# Autodesk Inventor assembly: Flex
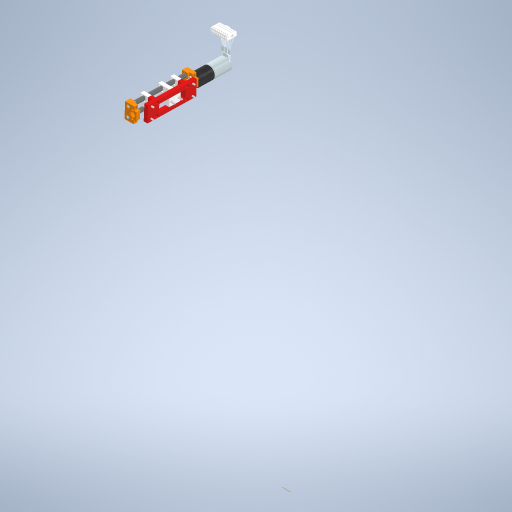
[picture p0: Inventor's stored thumbnail of the model, 512x512]
Saved by Autodesk Inventor 2023 (Build 270158000, 158)
## iProperties
Created: 2023-03-17
Part Number: Flex
Document SubType Name: Assembly
Designer: Nathann
Author: Nathann
## Documents named in this file (23)
- C:\Users\Nathann\ClawdDrive\Objet3D\IminaProbe\V3Roue\DifferentialLinearActuator.iam
- C:\Users\Nathann\OneDrive\ClawdDrive\Objet3D\IminaProbe\V2\Part1.ipt
- C:\Users\Nathann\OneDrive\ClawdDrive\Objet3D\IminaProbe\V2\GP16A_2-Stufig-110322.ipt
- C:\Users\Nathann\OneDrive\ClawdDrive\Objet3D\IminaProbe\V2\283825_ec-max16_5w.ipt
- C:\Users\Nathann\OneDrive\ClawdDrive\Objet3D\IminaProbe\V2\4145N198_Set Screw Precision Flexible Shaft Couplings.ipt
- C:\Users\Nathann\OneDrive\ClawdDrive\Objet3D\IminaProbe\V2\94450A564_Left-Hand Threaded 18-8 Stainless Steel Thin Hex Nut.ipt
- C:\Users\Nathann\OneDrive\ClawdDrive\Objet3D\IminaProbe\V2\91292A832_18-8 Stainless Steel Socket Head Screw.ipt
- C:\Users\Nathann\OneDrive\ClawdDrive\Objet3D\IminaProbe\V2\POMSliderMotor.ipt
- C:\Users\Nathann\OneDrive\ClawdDrive\Objet3D\IminaProbe\V2\MotorMountDifferential.ipt
- C:\Users\Nathann\OneDrive\ClawdDrive\Objet3D\IminaProbe\V2\93805A627_18-8 Stainless Steel Threaded Rod.ipt
- C:\Users\Nathann\OneDrive\ClawdDrive\Objet3D\IminaProbe\V2\93805A631_18-8 Stainless Steel Threaded Rod.ipt
- C:\Users\Nathann\OneDrive\ClawdDrive\Objet3D\IminaProbe\V2\91828A113_18-8 Stainless Steel Hex Nut.ipt
- C:\Users\Nathann\OneDrive\ClawdDrive\Objet3D\IminaProbe\V2\MotorDifferentialMountingBracket.ipt
- C:\Users\Nathann\OneDrive\ClawdDrive\Objet3D\IminaProbe\V2\POMSliderMotorM25.ipt
- C:\Users\Nathann\OneDrive\ClawdDrive\Objet3D\IminaProbe\V2\SliderFixtureM25.ipt
- C:\Users\Nathann\OneDrive\ClawdDrive\Objet3D\IminaProbe\V2\AxisLinear.ipt
- C:\Users\Nathann\OneDrive\ClawdDrive\Objet3D\IminaProbe\V2\POMSliderAxis.ipt
- C:\Users\Nathann\OneDrive\ClawdDrive\Objet3D\IminaProbe\V2\Flex\AIP\FEA\ea0gbbme8.fins
- C:\Users\Nathann\OneDrive\ClawdDrive\Objet3D\IminaProbe\V2\Flex\AIP\FEA\ea0gbbme8.fsat
- C:\Users\Nathann\OneDrive\ClawdDrive\Objet3D\IminaProbe\V2\Flex\AIP\FEA\ea0gbbme8.ftes
- C:\Users\Nathann\OneDrive\ClawdDrive\Objet3D\IminaProbe\V2\Flex\AIP\FEA\ea0gbbme8.fwiz
- C:\Users\Nathann\OneDrive\ClawdDrive\Objet3D\IminaProbe\V2\Flex\AIP\FEA\ea0gbbmf4.fmsh
- C:\Users\Nathann\OneDrive\ClawdDrive\Objet3D\IminaProbe\V2\Flex\AIP\FEA\ea0gbbmf5.fres
## Components (39 placed, 16 different names)
1. Part1:1
2. GP16A_2-Stufig-110322:2 — Insert:23, Insert:24
3. 283825_ec-max16_5w:2
4. 4145N198_Set Screw Precision Flexible Shaft Couplings:2 — Insert:27
5. 91292A832_18-8 Stainless Steel Socket Head Screw:5 — Insert:28
6. 91292A832_18-8 Stainless Steel Socket Head Screw:6 — Insert:29
7. MotorMountDifferential:1 — Insert:23, Insert:24, Insert:28, Insert:29, Flush:10, Flush:12, Flush:13, Insert:43, Insert:44, Insert:45, Insert:46
8. 93805A627_18-8 Stainless Steel Threaded Rod:1 — Insert:26, Rotation:1
9. 93805A631_18-8 Stainless Steel Threaded Rod:2 — Insert:26, Insert:27, Rotation:1
10. 91828A113_18-8 Stainless Steel Hex Nut:1 — Mate:26, Mate:27, Mate:28
11. 94450A564_Left-Hand Threaded 18-8 Stainless Steel Thin Hex Nut:3 — Mate:21, Mate:22, Mate:23
12. MotorDifferentialMountingBracket:1 — Insert:30, Insert:31, Insert:32, Insert:33, Flush:14, Flush:15, Mate:25, Insert:34, Insert:35, Insert:36, Insert:37, Flush:16, Mate:29, Flush:17
13. POMSliderMotorM25:1 — Mate:15, Flush:9, Flush:10, Flush:11, Mate:26, Mate:27, Mate:28, Insert:52, Flush:26
14. SliderFixtureM25:1 — Mate:15, Flush:9, Flush:11, Insert:38, Insert:39, Flush:17
15. POMSliderMotor:3 — Flush:12, Flush:14, Flush:15, Mate:25, Insert:53
16. POMSliderMotor:4 — Flush:13, Mate:21, Mate:22, Mate:23, Flush:16, Mate:29, Insert:51
17. 91292A832_18-8 Stainless Steel Socket Head Screw:9 — Insert:31
18. 91292A832_18-8 Stainless Steel Socket Head Screw:10 — Insert:30
19. 91292A832_18-8 Stainless Steel Socket Head Screw:11 — Insert:33
20. 91292A832_18-8 Stainless Steel Socket Head Screw:12 — Insert:32
21. 91292A832_18-8 Stainless Steel Socket Head Screw:13 — Insert:36
22. 91292A832_18-8 Stainless Steel Socket Head Screw:14 — Insert:34
23. 91292A832_18-8 Stainless Steel Socket Head Screw:15 — Insert:37
24. 91292A832_18-8 Stainless Steel Socket Head Screw:16 — Insert:35
25. 91292A832_18-8 Stainless Steel Socket Head Screw:17 — Insert:39
26. 91292A832_18-8 Stainless Steel Socket Head Screw:18 — Insert:38
27. AxisLinear:1 — Insert:43, Insert:47
28. AxisLinear:2 — Insert:44, Insert:48
29. 91292A832_18-8 Stainless Steel Socket Head Screw:19 — Insert:46
30. 91292A832_18-8 Stainless Steel Socket Head Screw:20 — Insert:45
31. MotorMountDifferential:2 — Insert:47, Insert:48, Insert:49, Insert:50, Flush:18
32. 91292A832_18-8 Stainless Steel Socket Head Screw:21 — Insert:49
33. 91292A832_18-8 Stainless Steel Socket Head Screw:22 — Insert:50
34. POMSliderAxis:1 — Insert:52, Insert:55, Flush:26
35. POMSliderAxis:2 — Insert:53, Insert:56, Flush:18
36. POMSliderAxis:3 — Insert:51, Insert:54
37. 91292A832_18-8 Stainless Steel Socket Head Screw:23 — Insert:56
38. 91292A832_18-8 Stainless Steel Socket Head Screw:24 — Insert:55
39. 91292A832_18-8 Stainless Steel Socket Head Screw:25 — Insert:54
## Relationships (53: Insert 32, Flush 11, Mate 9, RelateRotation 1)
- [Insert]: GP16A_2-Stufig-110322:2 ↔ 283825_ec-max16_5w:2
- [Insert] (-4 mm): GP16A_2-Stufig-110322:2 ↔ 4145N198_Set Screw Precision Flexible Shaft Couplings:2
- Insert:23: GP16A_2-Stufig-110322:2 ↔ MotorMountDifferential:1
- Insert:24: GP16A_2-Stufig-110322:2 ↔ MotorMountDifferential:1
- Insert:26: 93805A627_18-8 Stainless Steel Threaded Rod:1 ↔ 93805A631_18-8 Stainless Steel Threaded Rod:2
- Insert:27 (-4 mm): 4145N198_Set Screw Precision Flexible Shaft Couplings:2 ↔ 93805A631_18-8 Stainless Steel Threaded Rod:2
- Insert:28: 91292A832_18-8 Stainless Steel Socket Head Screw:5 ↔ MotorMountDifferential:1
- Insert:29: 91292A832_18-8 Stainless Steel Socket Head Screw:6 ↔ MotorMountDifferential:1
- Mate:15: POMSliderMotorM25:1 ↔ SliderFixtureM25:1
- Flush:9: POMSliderMotorM25:1 ↔ SliderFixtureM25:1
- Flush:10: MotorMountDifferential:1 ↔ POMSliderMotorM25:1
- Flush:11: POMSliderMotorM25:1 ↔ SliderFixtureM25:1
- Flush:12: MotorMountDifferential:1 ↔ POMSliderMotor:3
- Flush:13: MotorMountDifferential:1 ↔ POMSliderMotor:4
- Mate:21: 94450A564_Left-Hand Threaded 18-8 Stainless Steel Thin Hex Nut:3 ↔ POMSliderMotor:4
- Mate:22: 94450A564_Left-Hand Threaded 18-8 Stainless Steel Thin Hex Nut:3 ↔ POMSliderMotor:4
- Mate:23: 94450A564_Left-Hand Threaded 18-8 Stainless Steel Thin Hex Nut:3 ↔ POMSliderMotor:4
- Insert:30: MotorDifferentialMountingBracket:1 ↔ 91292A832_18-8 Stainless Steel Socket Head Screw:10
- Insert:31: MotorDifferentialMountingBracket:1 ↔ 91292A832_18-8 Stainless Steel Socket Head Screw:9
- Insert:32: MotorDifferentialMountingBracket:1 ↔ 91292A832_18-8 Stainless Steel Socket Head Screw:12
- Insert:33: MotorDifferentialMountingBracket:1 ↔ 91292A832_18-8 Stainless Steel Socket Head Screw:11
- Flush:14: MotorDifferentialMountingBracket:1 ↔ POMSliderMotor:3
- Flush:15: MotorDifferentialMountingBracket:1 ↔ POMSliderMotor:3
- Mate:25: MotorDifferentialMountingBracket:1 ↔ POMSliderMotor:3
- Insert:34: MotorDifferentialMountingBracket:1 ↔ 91292A832_18-8 Stainless Steel Socket Head Screw:14
- Insert:35: MotorDifferentialMountingBracket:1 ↔ 91292A832_18-8 Stainless Steel Socket Head Screw:16
- Insert:36: MotorDifferentialMountingBracket:1 ↔ 91292A832_18-8 Stainless Steel Socket Head Screw:13
- Insert:37: MotorDifferentialMountingBracket:1 ↔ 91292A832_18-8 Stainless Steel Socket Head Screw:15
- Flush:16: MotorDifferentialMountingBracket:1 ↔ POMSliderMotor:4
- Insert:38: SliderFixtureM25:1 ↔ 91292A832_18-8 Stainless Steel Socket Head Screw:18
- Insert:39: SliderFixtureM25:1 ↔ 91292A832_18-8 Stainless Steel Socket Head Screw:17
- Mate:26: 91828A113_18-8 Stainless Steel Hex Nut:1 ↔ POMSliderMotorM25:1
- Mate:27: 91828A113_18-8 Stainless Steel Hex Nut:1 ↔ POMSliderMotorM25:1
- Mate:28: 91828A113_18-8 Stainless Steel Hex Nut:1 ↔ POMSliderMotorM25:1
- Rotation:1 [RelateRotation] (1 ul): 93805A627_18-8 Stainless Steel Threaded Rod:1 ↔ 93805A631_18-8 Stainless Steel Threaded Rod:2
- Insert:43: MotorMountDifferential:1 ↔ AxisLinear:1
- Insert:44: MotorMountDifferential:1 ↔ AxisLinear:2
- Insert:45: MotorMountDifferential:1 ↔ 91292A832_18-8 Stainless Steel Socket Head Screw:20
- Insert:46: MotorMountDifferential:1 ↔ 91292A832_18-8 Stainless Steel Socket Head Screw:19
- Insert:47: AxisLinear:1 ↔ MotorMountDifferential:2
- Insert:48: AxisLinear:2 ↔ MotorMountDifferential:2
- Insert:49: MotorMountDifferential:2 ↔ 91292A832_18-8 Stainless Steel Socket Head Screw:21
- Insert:50: MotorMountDifferential:2 ↔ 91292A832_18-8 Stainless Steel Socket Head Screw:22
- Mate:29: MotorDifferentialMountingBracket:1 ↔ POMSliderMotor:4
- Insert:51: POMSliderMotor:4 ↔ POMSliderAxis:3
- Insert:52: POMSliderMotorM25:1 ↔ POMSliderAxis:1
- Insert:53: POMSliderMotor:3 ↔ POMSliderAxis:2
- Insert:54: POMSliderAxis:3 ↔ 91292A832_18-8 Stainless Steel Socket Head Screw:25
- Insert:55: POMSliderAxis:1 ↔ 91292A832_18-8 Stainless Steel Socket Head Screw:24
- Insert:56: POMSliderAxis:2 ↔ 91292A832_18-8 Stainless Steel Socket Head Screw:23
- Flush:17: MotorDifferentialMountingBracket:1 ↔ SliderFixtureM25:1
- Flush:18: MotorMountDifferential:2 ↔ POMSliderAxis:2
- Flush:26: POMSliderMotorM25:1 ↔ POMSliderAxis:1
## Named parameters: sa_0 = 1, d33_d3 = 0 mm, d43_d9 = -4 mm
note: some values were not read from the file. Shown as the stored number, unit unknown: "sa_0".
